# Autodesk Inventor assembly: Groove_Mount_Adaptor_1_75
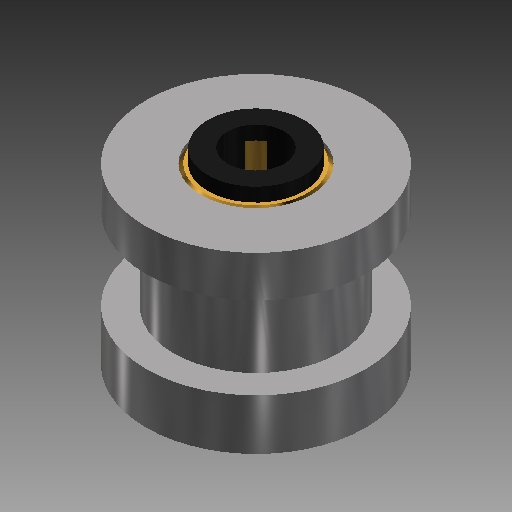
[picture p0: Inventor's stored thumbnail of the model, 512x512]
Saved by Autodesk Inventor 2019 (Build 230136000, 136)
## iProperties
Created: 2018-09-16
Part Number: Groove_Mount_Adaptor_1_75
Document SubType Name: Assembly
Designer: Ax
Author: Ax
## Documents named in this file (3)
- C:\Users\Ax\Google Drive\Inventor\Library\Drakon\Groove_Mount_Adaptor_1_75.iam
- C:\Users\Ax\Google Drive\Inventor\Library\Drakon\Groove_Mount_Adaptor_1_75mm.ipt
- C:\Users\Ax\Google Drive\Inventor\Library\Collet.ipt
## Components (2 placed, 2 different names)
1. Groove_Mount_Adaptor_1_75mm:1 — Flush:1, Mate:1
2. Collet:1 — Flush:1, Mate:1
## Relationships (2: Flush 1, Mate 1)
- Flush:1: Groove_Mount_Adaptor_1_75mm:1 ↔ Collet:1
- Mate:1: Groove_Mount_Adaptor_1_75mm:1 ↔ Collet:1
